# Autodesk Inventor assembly: 4. ALL_bez_Front
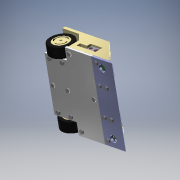
[picture p0: Inventor's stored thumbnail of the model, 180x180]
Saved by Autodesk Inventor 2017 (Build 210142000, 142)
## iProperties
Created: 2016-11-21
Part Number: 4. ALL_bez_Front
Document SubType Name: Assembly
Designer: Shichi
Author: Shichi
## Documents named in this file (5)
- E:\h3fty\H3FTY\Model\4. ALL_bez_Front.iam
- E:\h3fty\H3FTY\Model\PCB\PCB_2.ipt
- E:\h3fty\H3FTY\Model\3. P+K+O+PCB+Bateria.iam
- C:\Users\Shichi\Documents\Inventor\Content Center Files\R2017\en-US\AS 1112 (2)\AS 1112 - M2,5  Type 5.ipt
- E:\h3fty\H3FTY\Model\Inne\Podkladka_5mm.ipt
## Components (6 placed, 4 different names)
1. 3. P+K+O+PCB+Bateria:1 [sub-assembly] — Insert:1, Insert:4
2. Podkladka_5mm:1 — Insert:1, Insert:2
3. Podkladka_5mm:2 — Insert:2, Insert:3
4. PCB_2:1 — Insert:3, Insert:4, Insert:5, Insert:6
5. AS 1112 (2) - Metric M2,5  Type 5:1 — Insert:5
6. AS 1112 (2) - Metric M2,5  Type 5:2 — Insert:6
## Relationships (6: Insert 6)
- Insert:1: 3. P+K+O+PCB+Bateria:1 ↔ Podkladka_5mm:1
- Insert:2: Podkladka_5mm:1 ↔ Podkladka_5mm:2
- Insert:3: Podkladka_5mm:2 ↔ PCB_2:1
- Insert:4: 3. P+K+O+PCB+Bateria:1 ↔ PCB_2:1
- Insert:5: PCB_2:1 ↔ AS 1112 (2) - Metric M2,5  Type 5:1
- Insert:6: PCB_2:1 ↔ AS 1112 (2) - Metric M2,5  Type 5:2
